# Autodesk Inventor assembly: Skid Packaging Layout
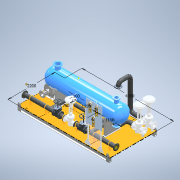
[picture p0: Inventor's stored thumbnail of the model, 180x180]
Saved by Autodesk Inventor 2020 (Build 240168000, 168)
## iProperties
RuleStatus: InUse
Created: 2009-08-05
Part Number: Skid Packaging Layout
Document SubType Name: Assembly
Designer: Demir Ali
Mass: 3.10272e+06 g
Surface Area: 859706 cm^2
Volume: 451428 cm^3
Density: 6.87311 g/cm^3
_SolveAssemblyDoc: Frame Generator Solve Assembly
_Version: 15.0.0
Author: Demir Ali
## Documents named in this file (15)
- C:\Dev\UpdateBom\UpdateBom\DebugPluginLocally\inputFiles\Process Equipment\Workspace\Skid Packaging Layout.iam
- C:\Dev\UpdateBom\UpdateBom\DebugPluginLocally\inputFiles\Process Equipment\Workspace\Framework\SV-Frame-Ref.ipt
- C:\Dev\UpdateBom\UpdateBom\DebugPluginLocally\inputFiles\Process Equipment\Workspace\Framework\SV-Frame-Assembly.iam
- C:\Dev\UpdateBom\UpdateBom\DebugPluginLocally\inputFiles\Process Equipment\Workspace\Components\AIP\Tube and Pipe\Seperator Vessel Layout.Tube and Pipe Runs.iam
- C:\Dev\UpdateBom\UpdateBom\DebugPluginLocally\inputFiles\Process Equipment\Workspace\Options\Pipe Support U-Ring.ipt
- C:\Dev\UpdateBom\UpdateBom\DebugPluginLocally\inputFiles\Process Equipment\Workspace\Options\Skid Lifting Plate.ipt
- C:\Dev\UpdateBom\UpdateBom\DebugPluginLocally\inputFiles\Process Equipment\Workspace\Options\Pipe Support Valve U-Ring.ipt
- C:\Dev\UpdateBom\UpdateBom\DebugPluginLocally\inputFiles\Process Equipment\Workspace\Supplier Content\Valves\Pipe Support U-Ring DN125.ipt
- C:\Dev\UpdateBom\UpdateBom\DebugPluginLocally\inputFiles\Process Equipment\Workspace\Options\Vessel Support A.ipt
- C:\Dev\UpdateBom\UpdateBom\DebugPluginLocally\inputFiles\Process Equipment\Workspace\Options\Vessel Support B.ipt
- C:\Dev\UpdateBom\UpdateBom\DebugPluginLocally\inputFiles\Process Equipment\Workspace\Options\Level Gauge Assembly.iam
- C:\Dev\UpdateBom\UpdateBom\DebugPluginLocally\inputFiles\Process Equipment\Workspace\Options\Sampling Connections.iam
- C:\Dev\UpdateBom\UpdateBom\DebugPluginLocally\inputFiles\Process Equipment\Workspace\Options\Instrumentation Panel.iam
- C:\Dev\UpdateBom\UpdateBom\DebugPluginLocally\inputFiles\Process Equipment\Workspace\Options\HSV-AD-B.ipt
- C:\Dev\UpdateBom\UpdateBom\DebugPluginLocally\inputFiles\Process Equipment\Workspace\Options\Pump Set.iam
## Components (26 placed, 14 different names)
1. Skid Plate — Flush:1, Flush:2, Flush:3, Rigid:2, Rigid:3, Rigid:4, Rigid:5, FlushV:28, FlushV:28_XZ, FlushV:28_YZ, MateV:33, MateV:34, FlushSp:8, FlushSp:9, MateSp:3, FlushSp:5, FlushSp:6, FlushSp:7, Flush:4, Flush:4_XZ, Flush:4_YZ
2. Skid Frame [sub-assembly]
3. Tube & Pipe Runs [sub-assembly]
4. Vessel — FlushV:28, FlushV:28_XZ, FlushV:28_YZ, FlushV:27, FlushV:37, FlushV:24, FlushV:25, InsertG:1, AngleG:1
5. Vessel Support A — FlushV:27, FlushV:37, MateV:33
6. Vessel Support B — FlushV:24, FlushV:25, MateV:34
7. Level Gauge Assembly [sub-assembly] — InsertG:1, AngleG:1
8. Sampling Connections [sub-assembly] — FlushSp:8, FlushSp:9, MateSp:3
9. Instrumentation Panel [sub-assembly] — FlushSp:5, FlushSp:6, FlushSp:7
10. Pump Set:1 [sub-assembly] — Flush:4, Flush:4_XZ, Flush:4_YZ
11. Pipe Support U-Ring:1 — Rigid:2
12. Pipe Support U-Ring:7
13. Pipe Support U-Ring:8
14. Pipe Support U-Ring:2
15. Pipe Support U-Ring:9
16. Pipe Support U-Ring:10
17. Pipe Support Valve U-Ring:1 — Rigid:4
18. Pipe Support Valve U-Ring:2
19. Pipe Support Valve U-Ring:3
20. Pipe Support Valve U-Ring:4
21. Pipe Support U-Ring DN125:1 — Rigid:5
22. Pipe Support U-Ring DN125:2
23. Skid Lifting Plate — Rigid:3
24. Skid Lifting Plate:2
25. Skid Lifting Plate:3
26. Skid Lifting Plate:4
## Component patterns: (6 elements, first: Pipe Support U-Ring:1), (4 elements, first: Pipe Support Valve U-Ring:1), (2 elements), (2 elements, first: Pipe Support U-Ring DN125:1), (2 elements, first: Skid Lifting Plate), Component Pattern 6:2 (2 elements)
## Relationships (27: Flush 18, WeldJoint 4, Mate 3, Insert 1, Angle 1)
- Flush:1: Skid Plate
- Flush:2: Skid Plate
- Flush:3 (2050 mm): Skid Plate
- Rigid:2 [WeldJoint]: Skid Plate ↔ Pipe Support U-Ring:1
- Rigid:3 [WeldJoint]: Skid Plate ↔ Skid Lifting Plate
- Rigid:4 [WeldJoint] (90 mm): Skid Plate ↔ Pipe Support Valve U-Ring:1
- Rigid:5 [WeldJoint]: Skid Plate ↔ Pipe Support U-Ring DN125:1
- FlushV:28 (-950 mm): Skid Plate ↔ Vessel
- FlushV:28_XZ: Skid Plate ↔ Vessel
- FlushV:28_YZ: Skid Plate ↔ Vessel
- FlushV:27: Vessel ↔ Vessel Support A
- FlushV:37 (1150 mm): Vessel ↔ Vessel Support A
- MateV:33: Skid Plate ↔ Vessel Support A
- FlushV:24: Vessel ↔ Vessel Support B
- FlushV:25 (-1150 mm): Vessel ↔ Vessel Support B
- MateV:34: Skid Plate ↔ Vessel Support B
- InsertG:1: Vessel ↔ Level Gauge Assembly
- AngleG:1 (180 deg): Vessel ↔ Level Gauge Assembly
- FlushSp:8 (-950 mm): Skid Plate ↔ Sampling Connections
- FlushSp:9 (525 mm): Skid Plate ↔ Sampling Connections
- MateSp:3 (-150 mm): Skid Plate ↔ Sampling Connections
- FlushSp:5: Skid Plate ↔ Instrumentation Panel
- FlushSp:6 (-1400 mm): Skid Plate ↔ Instrumentation Panel
- FlushSp:7 (1050 mm): Skid Plate ↔ Instrumentation Panel
- Flush:4: Skid Plate ↔ Pump Set:1
- Flush:4_XZ: Skid Plate ↔ Pump Set:1
- Flush:4_YZ (1750 mm): Skid Plate ↔ Pump Set:1
## Named parameters: iTrigger0 = 7, VesselOffset = 0 mm, PlateAngle = 125 deg
